# Autodesk Inventor assembly: ASSY_REV,ENG_DESIGN2
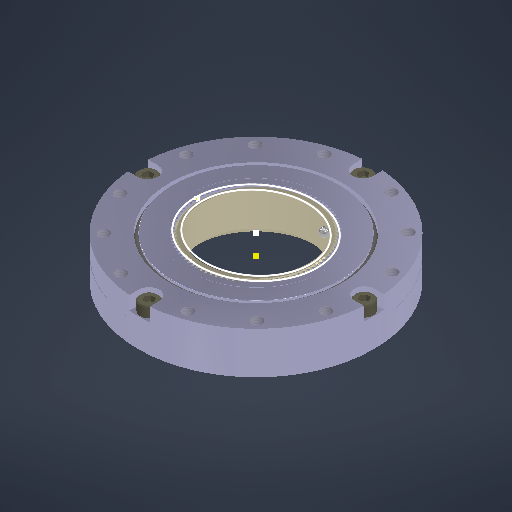
[picture p0: Inventor's stored thumbnail of the model, 512x512]
Saved by Autodesk Inventor 2026.2 (Build 302298010, 298A)
## iProperties
Created: 2026-02-10
Part Number: ASSY_REV,ENG_DESIGN2
Document SubType Name: Assembly
Designer: 4aida
Author: 4aida
## Documents named in this file (12)
- C:\Users\4aida\OneDrive\Documents\GitHub\Design_II_Group6\REV_ENG\ASSY_REV,ENG_DESIGN2.iam
- C:\Users\4aida\OneDrive\Documents\GitHub\Design_II_Group6\REV_ENG\ROLLER_CR_BEARING,REV-ENG.ipt
- C:\Users\4aida\OneDrive\Documents\GitHub\Design_II_Group6\REV_ENG\SPACER_ROLLER_CR_BEARING,REV-ENG.ipt
- C:\Users\4aida\OneDrive\Documents\GitHub\Design_II_Group6\REV_ENG\MIR_SPACER_ROLLER_CR_BEARING,REV-ENG.ipt
- C:\Users\4aida\OneDrive\Documents\GitHub\Design_II_Group6\REV_ENG\CR_ROLLER_BOUNDRY,REV-ENG.ipt
- C:\Users\4aida\OneDrive\Documents\GitHub\Design_II_Group6\REV_ENG\O_RING.ipt
- C:\Users\4aida\OneDrive\Documents\GitHub\Design_II_Group6\REV_ENG\CR_OUTSIDE,BOTTOM,REV-ENG.ipt
- C:\Users\4aida\OneDrive\Documents\GitHub\Design_II_Group6\REV_ENG\CR_OUTSIDE,TOP,REV-ENG.ipt
- C:\Users\4aida\OneDrive\Documents\GitHub\Design_II_Group6\REV_ENG\Fasteners\M3\SCREW,SOCKET-HD,P,12_9,M03X0_5X10MM.ipt
- C:\Users\4aida\OneDrive\Documents\GitHub\Design_II_Group6\REV_ENG\2.5mm_BALL_BEARINGS.ipt
- C:\Users\4aida\OneDrive\Documents\GitHub\Design_II_Group6\REV_ENG\Flex_SPLINE,REV-ENG.iam
- C:\Users\4aida\OneDrive\Documents\GitHub\Design_II_Group6\REV_ENG\DERIVEN_CR_INSIDE,REV-ENG.ipt
## Components (59 placed, 11 different names)
1. CR_ROLLER_BOUNDRY,REV-ENG:1 — Mate:23, Mate:24
2. O_RING:1 — Mate:16, Tangent:7
3. CR_OUTSIDE,BOTTOM,REV-ENG:1 — Mate:9, Mate:10, Mate:13, Flush:4, Mate:25
4. CR_OUTSIDE,TOP,REV-ENG:1 — Mate:9, Mate:10, Mate:12, Flush:6, Mate:17, Insert:1, Insert:2, Insert:3, Insert:4
5. SCREW,SOCKET-HD,P,12_9,M03X0_5X10MM:1 — Insert:1
6. 2.5mm_BALL_BEARINGS:1 — Tangent:5, Tangent:6
7. Flex_SPLINE,REV-ENG:1 [sub-assembly] — Tangent:5, Tangent:6, Flush:5, Mate:15, Mate:25
8. DERIVEN_CR_INSIDE,REV-ENG:1 — Flush:5, Mate:15, Mate:16, Tangent:7, Flush:6, Mate:17, Mate:18, Mate:21, Tangent:8, Tangent:9
9. SCREW,SOCKET-HD,P,12_9,M03X0_5X10MM:2 — Insert:4
10. SCREW,SOCKET-HD,P,12_9,M03X0_5X10MM:3 — Insert:2
11. SCREW,SOCKET-HD,P,12_9,M03X0_5X10MM:4 — Insert:3
12. MIR_SPACER_ROLLER_CR_BEARING,REV-ENG:13 — Mate:21, Mate:22
13. ROLLER_CR_BEARING,REV-ENG:27 — Mate:20, Mate:22, Tangent:8
14. SPACER_ROLLER_CR_BEARING,REV-ENG:13 — Mate:18, Mate:19, Flush:7, Mate:20
15. ROLLER_CR_BEARING,REV-ENG:26 — Mate:19, Tangent:9
16. MIR_SPACER_ROLLER_CR_BEARING,REV-ENG:14
17. ROLLER_CR_BEARING,REV-ENG:28
18. SPACER_ROLLER_CR_BEARING,REV-ENG:14
19. ROLLER_CR_BEARING,REV-ENG:29
20. MIR_SPACER_ROLLER_CR_BEARING,REV-ENG:15
21. ROLLER_CR_BEARING,REV-ENG:30
22. SPACER_ROLLER_CR_BEARING,REV-ENG:15
23. ROLLER_CR_BEARING,REV-ENG:31
24. MIR_SPACER_ROLLER_CR_BEARING,REV-ENG:16
25. ROLLER_CR_BEARING,REV-ENG:32
26. SPACER_ROLLER_CR_BEARING,REV-ENG:16
27. ROLLER_CR_BEARING,REV-ENG:33
28. MIR_SPACER_ROLLER_CR_BEARING,REV-ENG:17
29. ROLLER_CR_BEARING,REV-ENG:34
30. SPACER_ROLLER_CR_BEARING,REV-ENG:17
31. ROLLER_CR_BEARING,REV-ENG:35
32. MIR_SPACER_ROLLER_CR_BEARING,REV-ENG:18
33. ROLLER_CR_BEARING,REV-ENG:36
34. SPACER_ROLLER_CR_BEARING,REV-ENG:18
35. ROLLER_CR_BEARING,REV-ENG:37
36. MIR_SPACER_ROLLER_CR_BEARING,REV-ENG:19
37. ROLLER_CR_BEARING,REV-ENG:38
38. SPACER_ROLLER_CR_BEARING,REV-ENG:19
39. ROLLER_CR_BEARING,REV-ENG:39
40. MIR_SPACER_ROLLER_CR_BEARING,REV-ENG:20
41. ROLLER_CR_BEARING,REV-ENG:40
42. SPACER_ROLLER_CR_BEARING,REV-ENG:20
43. ROLLER_CR_BEARING,REV-ENG:41
44. MIR_SPACER_ROLLER_CR_BEARING,REV-ENG:21
45. ROLLER_CR_BEARING,REV-ENG:42
46. SPACER_ROLLER_CR_BEARING,REV-ENG:21
47. ROLLER_CR_BEARING,REV-ENG:43
48. MIR_SPACER_ROLLER_CR_BEARING,REV-ENG:22
49. ROLLER_CR_BEARING,REV-ENG:44
50. SPACER_ROLLER_CR_BEARING,REV-ENG:22
51. ROLLER_CR_BEARING,REV-ENG:45
52. MIR_SPACER_ROLLER_CR_BEARING,REV-ENG:23
53. ROLLER_CR_BEARING,REV-ENG:46
54. SPACER_ROLLER_CR_BEARING,REV-ENG:23
55. ROLLER_CR_BEARING,REV-ENG:47
56. MIR_SPACER_ROLLER_CR_BEARING,REV-ENG:24
57. ROLLER_CR_BEARING,REV-ENG:48
58. SPACER_ROLLER_CR_BEARING,REV-ENG:24
59. ROLLER_CR_BEARING,REV-ENG:49
## Component patterns: (12 elements, first: MIR_SPACER_ROLLER_CR_BEARING,REV-ENG:13 + ROLLER_CR_BEARING,REV-ENG:27 + SPACER_ROLLER_CR_BEARING,REV-ENG:13 + ROLLER_CR_BEARING,REV-ENG:26)
## Relationships (28: Mate 15, Tangent 5, Flush 4, Insert 4)
- Mate:9: CR_OUTSIDE,BOTTOM,REV-ENG:1 ↔ CR_OUTSIDE,TOP,REV-ENG:1
- Mate:10: CR_OUTSIDE,BOTTOM,REV-ENG:1 ↔ CR_OUTSIDE,TOP,REV-ENG:1
- Tangent:5: 2.5mm_BALL_BEARINGS:1 ↔ Flex_SPLINE,REV-ENG:1
- Tangent:6: 2.5mm_BALL_BEARINGS:1 ↔ Flex_SPLINE,REV-ENG:1
- Mate:12: CR_OUTSIDE,TOP,REV-ENG:1
- Mate:13: CR_OUTSIDE,BOTTOM,REV-ENG:1
- Flush:4: CR_OUTSIDE,BOTTOM,REV-ENG:1
- Flush:5: Flex_SPLINE,REV-ENG:1 ↔ DERIVEN_CR_INSIDE,REV-ENG:1
- Mate:15: Flex_SPLINE,REV-ENG:1 ↔ DERIVEN_CR_INSIDE,REV-ENG:1
- Mate:16: O_RING:1 ↔ DERIVEN_CR_INSIDE,REV-ENG:1
- Tangent:7: O_RING:1 ↔ DERIVEN_CR_INSIDE,REV-ENG:1
- Flush:6: CR_OUTSIDE,TOP,REV-ENG:1 ↔ DERIVEN_CR_INSIDE,REV-ENG:1
- Mate:17: CR_OUTSIDE,TOP,REV-ENG:1 ↔ DERIVEN_CR_INSIDE,REV-ENG:1
- Mate:18: DERIVEN_CR_INSIDE,REV-ENG:1 ↔ SPACER_ROLLER_CR_BEARING,REV-ENG:13
- Mate:19: SPACER_ROLLER_CR_BEARING,REV-ENG:13 ↔ ROLLER_CR_BEARING,REV-ENG:26
- Flush:7: SPACER_ROLLER_CR_BEARING,REV-ENG:13
- Mate:20: ROLLER_CR_BEARING,REV-ENG:27 ↔ SPACER_ROLLER_CR_BEARING,REV-ENG:13
- Mate:21: DERIVEN_CR_INSIDE,REV-ENG:1 ↔ MIR_SPACER_ROLLER_CR_BEARING,REV-ENG:13
- Mate:22: MIR_SPACER_ROLLER_CR_BEARING,REV-ENG:13 ↔ ROLLER_CR_BEARING,REV-ENG:27
- Tangent:8 (0.125 mm): DERIVEN_CR_INSIDE,REV-ENG:1 ↔ ROLLER_CR_BEARING,REV-ENG:27
- Tangent:9 (0.125 mm): DERIVEN_CR_INSIDE,REV-ENG:1 ↔ ROLLER_CR_BEARING,REV-ENG:26
- Mate:23: CR_ROLLER_BOUNDRY,REV-ENG:1
- Mate:24: CR_ROLLER_BOUNDRY,REV-ENG:1
- Mate:25: CR_OUTSIDE,BOTTOM,REV-ENG:1 ↔ Flex_SPLINE,REV-ENG:1
- Insert:1: CR_OUTSIDE,TOP,REV-ENG:1 ↔ SCREW,SOCKET-HD,P,12_9,M03X0_5X10MM:1
- Insert:2: CR_OUTSIDE,TOP,REV-ENG:1 ↔ SCREW,SOCKET-HD,P,12_9,M03X0_5X10MM:3
- Insert:3: CR_OUTSIDE,TOP,REV-ENG:1 ↔ SCREW,SOCKET-HD,P,12_9,M03X0_5X10MM:4
- Insert:4: CR_OUTSIDE,TOP,REV-ENG:1 ↔ SCREW,SOCKET-HD,P,12_9,M03X0_5X10MM:2
